# Autodesk Inventor assembly: Leg
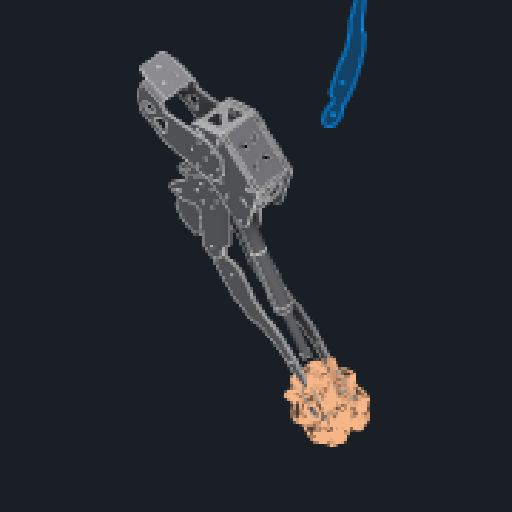
[picture p0: Inventor's stored thumbnail of the model, 512x512]
Saved by Autodesk Inventor 2025.2 (Build 292293000, 293)
## iProperties
Created: 2020-05-17
Part Number: Leg
Document SubType Name: Assembly
Designer: valer
Author: valer
## Documents named in this file (10)
- C:\Users\valer\Desktop\str1ker\cad\Leg.iam
- C:\Users\valer\Desktop\str1ker\cad\Knee.ipt
- C:\Users\valer\Desktop\str1ker\cad\LowerLeg.ipt
- C:\Users\valer\Desktop\str1ker\cad\UpperLeg.ipt
- C:\Users\valer\Desktop\str1ker\cad\Hip.ipt
- C:\Users\valer\Desktop\str1ker\cad\HipCoverTop.ipt
- C:\Users\valer\Desktop\str1ker\cad\external\MecanumWheel\Mecanum Wheel Derived.ipt
- C:\Users\valer\Desktop\str1ker\cad\external\TsinyMotorMY1016Z2_12VDC_300RPM_250W.ipt
- C:\Users\valer\Desktop\str1ker\cad\external\FA-RMS-15-12-4-Piston.ipt
- C:\Users\valer\Desktop\str1ker\cad\external\FA-RMS-15-12-4.ipt
## Components (12 placed, 9 different names)
1. Knee:1 — Flush:1, Mate:1, Mate:3, Mate:4, Mate:14
2. LowerLeg:1 — Mate:3, Mate:14, Mate:22, Mate:23, Mate:30
3. UpperLeg:1 — Flush:1, Mate:1, Mate:4, Mate:5, Mate:6, Mate:7, Mate:16, Mate:17, Mate:18, Mate:26, Symmetry:1
4. Hip:1 — Mate:5, Mate:6, Mate:7, Mate:12, Mate:13
5. Knee:2 — Mate:15, Mate:31
6. LowerLeg:2 — Mate:15, Mate:30, Mate:33
7. UpperLeg:2 — Mate:12, Mate:13, Symmetry:1, Mate:32
8. HipCoverTop:1 — Mate:16, Mate:17, Mate:18, Mate:32
9. Mecanum Wheel Derived:1 — Mate:22, Mate:23, Angle:3
10. TsinyMotorMY1016Z2_12VDC_300RPM_250W:1 — Mate:26
11. FA-RMS-15-12-4-Piston:1 — Mate:27, Angle:3, Mate:33
12. FA-RMS-15-12-4:1 — Mate:27, Flush:4, Mate:31
## Relationships (29: Mate 24, Flush 3, Symmetry 1, Angle 1)
- Flush:1 (-5.08 mm): Knee:1 ↔ UpperLeg:1
- Mate:1: Knee:1 ↔ UpperLeg:1
- Mate:3: Knee:1 ↔ LowerLeg:1
- Mate:4: Knee:1 ↔ UpperLeg:1
- Mate:5: UpperLeg:1 ↔ Hip:1
- Mate:6: UpperLeg:1 ↔ Hip:1
- Mate:7: UpperLeg:1 ↔ Hip:1
- [Flush] (5.08 mm): Knee:2 ↔ UpperLeg:2
- [Mate]: Knee:2 ↔ UpperLeg:2
- [Mate]: Knee:2 ↔ LowerLeg:2
- [Mate]: Knee:2 ↔ UpperLeg:2
- Mate:12: Hip:1 ↔ UpperLeg:2
- Mate:13: Hip:1 ↔ UpperLeg:2
- Mate:14: Knee:1 ↔ LowerLeg:1
- Mate:15: Knee:2 ↔ LowerLeg:2
- Mate:16: UpperLeg:1 ↔ HipCoverTop:1
- Mate:17: UpperLeg:1 ↔ HipCoverTop:1
- Mate:18: UpperLeg:1 ↔ HipCoverTop:1
- Mate:22: LowerLeg:1 ↔ Mecanum Wheel Derived:1
- Mate:23 (12.7 mm): LowerLeg:1 ↔ Mecanum Wheel Derived:1
- Mate:26 (10 mm): UpperLeg:1 ↔ TsinyMotorMY1016Z2_12VDC_300RPM_250W:1
- Mate:27: FA-RMS-15-12-4-Piston:1 ↔ FA-RMS-15-12-4:1
- Symmetry:1: UpperLeg:1 ↔ UpperLeg:2
- Flush:4: FA-RMS-15-12-4:1
- Angle:3 (0 deg): Mecanum Wheel Derived:1 ↔ FA-RMS-15-12-4-Piston:1
- Mate:30: LowerLeg:1 ↔ LowerLeg:2
- Mate:31: Knee:2 ↔ FA-RMS-15-12-4:1
- Mate:32: UpperLeg:2 ↔ HipCoverTop:1
- Mate:33: LowerLeg:2 ↔ FA-RMS-15-12-4-Piston:1
## Named parameters: d11_d0 = 5.08 mm, d12_d1 = 0 mm, d14_d4 = 0 mm, d15_d5 = 0 mm
